# Autodesk Inventor assembly: controlbox
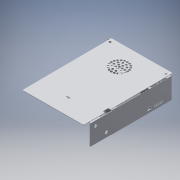
[picture p0: Inventor's stored thumbnail of the model, 180x180]
Saved by Autodesk Inventor 2017 (Build 210142000, 142)
## iProperties
Created: 2018-07-05
Part Number: controlbox
Document SubType Name: Assembly
Designer: UnKnoWn
Author: UnKnoWn
## Documents named in this file (4)
- I:\3d Printer stuff\Ender 3\Ender3 working files\Ender-3 Mechanical\STP\controlbox.iam
- I:\3d Printer stuff\Ender 3\Ender3 working files\Ender-3 Mechanical\STP\Sheetmetal enclosure bottom.ipt
- I:\3d Printer stuff\Ender 3\Ender3 working files\Ender-3 Mechanical\STP\Sheetmetal enclosure top.ipt
- I:\3d Printer stuff\Ender 3\Ender3 working files\Ender-3 Mechanical\STP\Control panel.ipt
## Components (3 placed, 3 different names)
1. Sheetmetal enclosure bottom:1 — Mate:1, Mate:2, Mate:3
2. Sheetmetal enclosure top:1 — Mate:1
3. Control panel:1 — Mate:2, Mate:3
## Relationships (3: Mate 3)
- Mate:1: Sheetmetal enclosure bottom:1 ↔ Sheetmetal enclosure top:1
- Mate:2: Sheetmetal enclosure bottom:1 ↔ Control panel:1
- Mate:3: Sheetmetal enclosure bottom:1 ↔ Control panel:1
